# Autodesk Inventor assembly: Zusammenbau
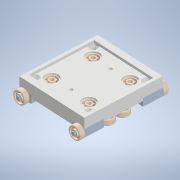
[picture p0: Inventor's stored thumbnail of the model, 180x180]
Saved by Autodesk Inventor 2022 (Build 260153000, 153)
## iProperties
Created: 2022-04-21
Part Number: Zusammenbau
Document SubType Name: Assembly
Designer: 123St
Author: 123St
## Documents named in this file (5)
- C:\Users\alexw\Documents\Inventor\Projects\03_CurrentProjects\MasterThesis\PSM_V1_Rillenkugellager\Ueberarbeiteter DaVincikopf\Zusammenbau.iam
- C:\Users\alexw\Documents\Inventor\Projects\03_CurrentProjects\MasterThesis\PSM_V1_Rillenkugellager\Ueberarbeiteter DaVincikopf\Fuehrungsgrundplatte.ipt
- C:\Users\alexw\Documents\Inventor\Projects\03_CurrentProjects\MasterThesis\PSM_V1_Rillenkugellager\Ueberarbeiteter DaVincikopf\Fuehrungslagerhalter_v1.ipt
- C:\Users\alexw\Documents\Inventor\Projects\03_CurrentProjects\MasterThesis\PSM_V1_Rillenkugellager\Ueberarbeiteter DaVincikopf\126017015-9-bb-623-a500-70-es\bb-623-a500-70-es.iam
- C:\Users\alexw\Documents\Inventor\Projects\03_CurrentProjects\MasterThesis\PSM_V1_Rillenkugellager\Ueberarbeiteter DaVincikopf\Lagerhalterung.ipt
## Components (16 placed, 4 different names)
1. Fuehrungsgrundplatte:1 — Passend:1, Passend:2, Passend:3, Passend:4, Einfügen:1, Einfügen:2, Einfügen:3, Einfügen:4, Einfügen:5, Einfügen:6, Einfügen:7, Einfügen:8
2. Fuehrungslagerhalter_v1:1 — Passend:2, Passend:4, Einfügen:1, Drehbar:5, Drehbar:8, Drehbar:11, Drehbar:12
3. Fuehrungslagerhalter_v1:2 — Passend:1, Passend:3, Einfügen:2, Drehbar:2, Drehbar:3, Drehbar:9, Drehbar:10
4. bb-623-a500-70-es:1 [sub-assembly] — Drehbar:2
5. bb-623-a500-70-es:2 [sub-assembly] — Drehbar:9
6. bb-623-a500-70-es:3 [sub-assembly] — Drehbar:10
7. bb-623-a500-70-es:4 [sub-assembly] — Drehbar:3
8. bb-623-a500-70-es:5 [sub-assembly] — Drehbar:5
9. bb-623-a500-70-es:6 [sub-assembly] — Drehbar:8
10. bb-623-a500-70-es:7 [sub-assembly] — Drehbar:12
11. bb-623-a500-70-es:8 [sub-assembly] — Drehbar:11
12. Lagerhalterung:1 — Einfügen:3, Einfügen:4
13. bb-623-a500-70-es:9 [sub-assembly] — Einfügen:5
14. bb-623-a500-70-es:10 [sub-assembly] — Einfügen:7
15. bb-623-a500-70-es:11 [sub-assembly] — Einfügen:8
16. bb-623-a500-70-es:12 [sub-assembly] — Einfügen:6
## Relationships (20: Insert 8, RevoluteJoint 8, Mate 4)
- Passend:1 [Mate]: Fuehrungsgrundplatte:1 ↔ Fuehrungslagerhalter_v1:2
- Passend:2 [Mate]: Fuehrungsgrundplatte:1 ↔ Fuehrungslagerhalter_v1:1
- Passend:3 [Mate]: Fuehrungsgrundplatte:1 ↔ Fuehrungslagerhalter_v1:2
- Passend:4 [Mate]: Fuehrungsgrundplatte:1 ↔ Fuehrungslagerhalter_v1:1
- Einfügen:1 [Insert]: Fuehrungsgrundplatte:1 ↔ Fuehrungslagerhalter_v1:1
- Einfügen:2 [Insert]: Fuehrungsgrundplatte:1 ↔ Fuehrungslagerhalter_v1:2
- Drehbar:2 [RevoluteJoint]: Fuehrungslagerhalter_v1:2 ↔ bb-623-a500-70-es:1
- Drehbar:3 [RevoluteJoint]: Fuehrungslagerhalter_v1:2 ↔ bb-623-a500-70-es:4
- Drehbar:5 [RevoluteJoint]: Fuehrungslagerhalter_v1:1 ↔ bb-623-a500-70-es:5
- Drehbar:8 [RevoluteJoint]: Fuehrungslagerhalter_v1:1 ↔ bb-623-a500-70-es:6
- Drehbar:9 [RevoluteJoint]: Fuehrungslagerhalter_v1:2 ↔ bb-623-a500-70-es:2
- Drehbar:10 [RevoluteJoint]: Fuehrungslagerhalter_v1:2 ↔ bb-623-a500-70-es:3
- Drehbar:11 [RevoluteJoint]: Fuehrungslagerhalter_v1:1 ↔ bb-623-a500-70-es:8
- Drehbar:12 [RevoluteJoint]: Fuehrungslagerhalter_v1:1 ↔ bb-623-a500-70-es:7
- Einfügen:3 [Insert]: Fuehrungsgrundplatte:1 ↔ Lagerhalterung:1
- Einfügen:4 [Insert]: Fuehrungsgrundplatte:1 ↔ Lagerhalterung:1
- Einfügen:5 [Insert]: Fuehrungsgrundplatte:1 ↔ bb-623-a500-70-es:9
- Einfügen:6 [Insert]: Fuehrungsgrundplatte:1 ↔ bb-623-a500-70-es:12
- Einfügen:7 [Insert]: Fuehrungsgrundplatte:1 ↔ bb-623-a500-70-es:10
- Einfügen:8 [Insert]: Fuehrungsgrundplatte:1 ↔ bb-623-a500-70-es:11
